# Autodesk Inventor assembly: excabadora
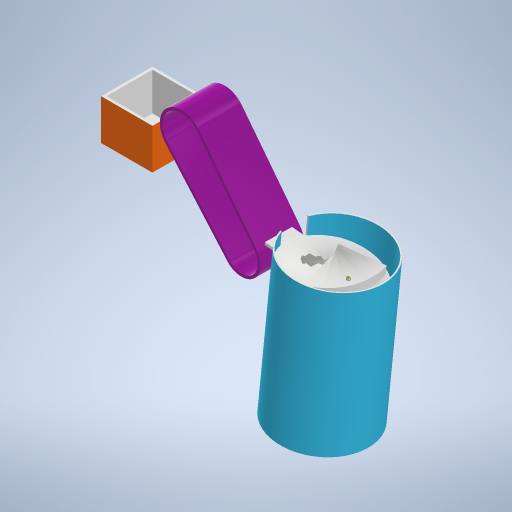
[picture p0: Inventor's stored thumbnail of the model, 512x512]
Saved by Autodesk Inventor 2023 (Build 270158000, 158)
## iProperties
Created: 2022-04-04
Part Number: excabadora
Document SubType Name: Assembly
Designer: isaac
Author: isaac
## Documents named in this file (5)
- C:\Users\isaac\OneDrive\Documentos\Diseño mecánico\excabadora.iam
- C:\Users\isaac\OneDrive\Documentos\Diseño mecánico\tuvo.ipt
- C:\Users\isaac\OneDrive\Documentos\Diseño mecánico\bobina.ipt
- C:\Users\isaac\OneDrive\Documentos\Diseño mecánico\banda.ipt
- C:\Users\isaac\OneDrive\Documentos\Diseño mecánico\cubo.ipt
## Components (4 placed, 4 different names)
1. banda:1 — De rotación:2
2. cubo:1
3. bobina:1 — De rotación:1
4. tuvo:1 — De rotación:1, De rotación:2
## Relationships (2: RevoluteJoint 2)
- De rotación:1 [RevoluteJoint]: bobina:1 ↔ tuvo:1
- De rotación:2 [RevoluteJoint]: banda:1 ↔ tuvo:1
